# Autodesk Inventor assembly: X_Führung
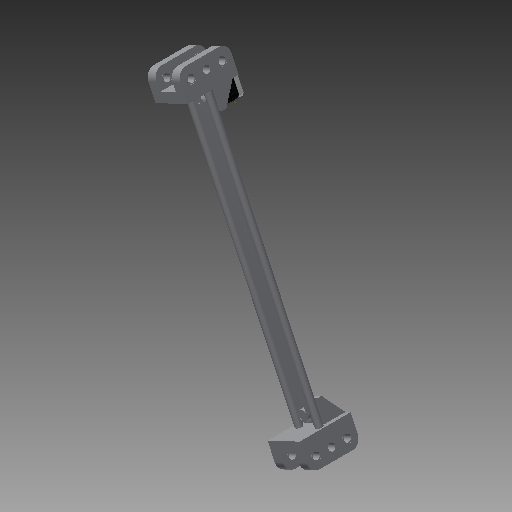
[picture p0: Inventor's stored thumbnail of the model, 512x512]
Saved by Autodesk Inventor 2019 (Build 230136000, 136)
## iProperties
Created: 2018-08-25
Part Number: X_Führung
Document SubType Name: Assembly
Designer: Julia
Author: Julia
## Documents named in this file (5)
- C:\Users\Julia\Documents\Inventor\3d_Drucker_v03_vertikaler_Gurt\X_Führung.iam
- C:\Users\Julia\Documents\Inventor\3d_Drucker_v03_vertikaler_Gurt\Y_Slider.iam
- C:\Users\Julia\Documents\Inventor\3d_Drucker_v03_vertikaler_Gurt\Y_Slider_mit_Schrittmotor.iam
- C:\Users\Julia\Documents\Inventor\3d_Drucker_v03_vertikaler_Gurt\X_Führungsstange.ipt
- C:\Users\Julia\Documents\Inventor\3d_Drucker_v03_vertikaler_Gurt\X_Zahnriemen.ipt
## Components (5 placed, 4 different names)
1. Y_Slider:1 [sub-assembly] — Mate:7, Mate:8, Mate:9, Angle:1, Angle:2, Flush:1, Mate:10
2. Y_Slider_mit_Schrittmotor:1 [sub-assembly] — Mate:1, Mate:2, Mate:3, Mate:4
3. X_Führungsstange:1 — Mate:1, Mate:3, Mate:7, Mate:9
4. X_Führungsstange:2 — Mate:2, Mate:4, Mate:8
5. X_Zahnriemen:1 — Angle:1, Angle:2, Flush:1, Mate:10
## Relationships (11: Mate 8, Angle 2, Flush 1)
- Mate:1: Y_Slider_mit_Schrittmotor:1 ↔ X_Führungsstange:1
- Mate:2: Y_Slider_mit_Schrittmotor:1 ↔ X_Führungsstange:2
- Mate:3: Y_Slider_mit_Schrittmotor:1 ↔ X_Führungsstange:1
- Mate:4: Y_Slider_mit_Schrittmotor:1 ↔ X_Führungsstange:2
- Mate:7: Y_Slider:1 ↔ X_Führungsstange:1
- Mate:8: Y_Slider:1 ↔ X_Führungsstange:2
- Mate:9: Y_Slider:1 ↔ X_Führungsstange:1
- Angle:1 (0 deg): Y_Slider:1 ↔ X_Zahnriemen:1
- Angle:2 (0 deg): Y_Slider:1 ↔ X_Zahnriemen:1
- Flush:1: Y_Slider:1 ↔ X_Zahnriemen:1
- Mate:10: Y_Slider:1 ↔ X_Zahnriemen:1
